# Autodesk Inventor assembly: arduino sitting
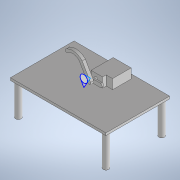
[picture p0: Inventor's stored thumbnail of the model, 180x180]
Saved by Autodesk Inventor 2020 (Build 240168000, 168)
## iProperties
Created: 2022-02-14
Part Number: arduino sitting
Document SubType Name: Assembly
Designer: rwte
Author: rwte
## Documents named in this file (3)
- C:\Users\chanc\Documents\GitHub\Dfab-AY21-22S2-Chan-Carl\CAD\final project\ipt files\arduino sitting.iam
- C:\Users\chanc\Documents\GitHub\Dfab-AY21-22S2-Chan-Carl\CAD\final project\ipt files\table top.ipt
- C:\Users\chanc\Documents\GitHub\Dfab-AY21-22S2-Chan-Carl\CAD\final project\ipt files\servo.ipt
## Components (2 placed, 2 different names)
1. table top:1 — Mate:1
2. servo:1 — Mate:1
## Relationships (1: Mate 1)
- Mate:1: table top:1 ↔ servo:1
